# Autodesk Inventor assembly: ASY GNH 010 Dilution point
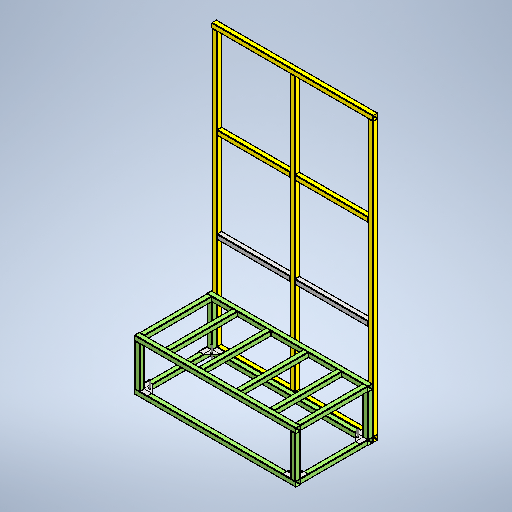
[picture p0: Inventor's stored thumbnail of the model, 512x512]
Saved by Autodesk Inventor 2025.1 (Build 291241020, 241B)
## iProperties
Created: 2025-03-06
Part Number: ASY GNH 010 Dilution point
Document SubType Name: Assembly
Designer: user
Author: user
## Documents named in this file (3)
- C:\Users\user\YandexDisk-badmisterfox\home pc\Inventor\GNH-Petrodvorec\ASY GNH 010 Dilution point.iam
- C:\Users\user\YandexDisk-badmisterfox\home pc\Inventor\GNH-Petrodvorec\ASY GNH 011 Dilution point Frame1.iam
- C:\Users\user\YandexDisk-badmisterfox\home pc\Inventor\GNH-Petrodvorec\ASY GNH 012 Dilution point Frame2.iam
## Components (2 placed, 2 different names)
1. ASY GNH 011 Dilution point Frame1:1 [sub-assembly]
2. ASY GNH 012 Dilution point Frame2:1 [sub-assembly]
## Relationships (1: WeldJoint 1)
- [WeldJoint]: ASY GNH 011 Dilution point Frame1:1 ↔ ASY GNH 012 Dilution point Frame2:1
